# Autodesk Inventor assembly: EntradaObert3
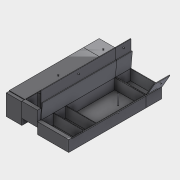
[picture p0: Inventor's stored thumbnail of the model, 180x180]
Saved by Autodesk Inventor 2022 (Build 260153000, 153)
## iProperties
Created: 2022-08-16
Part Number: EntradaObert3
Document SubType Name: Assembly
Designer: tesfa
Author: tesfa
## Documents named in this file (4)
- C:\Users\tesfa\Documents\XerracSA\segon\Entrada\EntradaObert3.iam
- C:\Users\tesfa\Documents\XerracSA\segon\Entrada\EntradaCentralObertMig.iam
- C:\Users\tesfa\Documents\XerracSA\segon\Entrada\EntradaDretaObert.iam
- C:\Users\tesfa\Documents\XerracSA\segon\Entrada\EntradaEsquerraTancat.iam
## Components (3 placed, 3 different names)
1. EntradaCentralObertMig:1 [sub-assembly] — Coincidencia:1, Nivelación:1, Nivelación:2, Coincidencia:2, Nivelación:3
2. EntradaDretaObert:1 [sub-assembly] — Coincidencia:2, Nivelación:3, Nivelación:4
3. EntradaEsquerraTancat:1 [sub-assembly] — Coincidencia:1, Nivelación:1, Nivelación:2, Nivelación:4
## Relationships (6: Flush 4, Mate 2)
- Coincidencia:1 [Mate]: EntradaCentralObertMig:1 ↔ EntradaEsquerraTancat:1
- Nivelación:1 [Flush]: EntradaCentralObertMig:1 ↔ EntradaEsquerraTancat:1
- Nivelación:2 [Flush]: EntradaCentralObertMig:1 ↔ EntradaEsquerraTancat:1
- Coincidencia:2 [Mate]: EntradaCentralObertMig:1 ↔ EntradaDretaObert:1
- Nivelación:3 [Flush]: EntradaCentralObertMig:1 ↔ EntradaDretaObert:1
- Nivelación:4 [Flush]: EntradaDretaObert:1 ↔ EntradaEsquerraTancat:1
